# Autodesk Inventor assembly: SumpAssembly
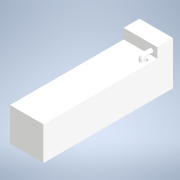
[picture p0: Inventor's stored thumbnail of the model, 180x180]
Saved by Autodesk Inventor 2022 (Build 260153000, 153)
## iProperties
Created: 2021-06-30
Part Number: SumpAssembly
Document SubType Name: Assembly
Designer: jamieson-bl
Author: jamieson-bl
## Documents named in this file (4)
- \\Mac\Home\Desktop\WinnipegPMTTestFacility\SumpAssembly.iam
- \\Mac\Home\Desktop\WinnipegPMTTestFacility\Sump_1SDB_Tub.ipt
- \\Mac\Home\Desktop\WinnipegPMTTestFacility\Sump Baffle Tub.ipt
- \\Mac\Home\Desktop\WinnipegPMTTestFacility\Sump Reservoir.ipt
## Components (4 placed, 3 different names)
1. Sump_1SDB_Tub:1 — Mate:1, Flush:1, Flush:2
2. Sump Baffle Tub:1 — Mate:1, Flush:1, Flush:2, Flush:3, Mate:2, Flush:5
3. Sump Reservoir:1 — Flush:3, Flush:4, Mate:2, Flush:5, Flush:6, Mate:3
4. Sump Reservoir:2 — Flush:4, Flush:6, Mate:3
## Relationships (9: Flush 6, Mate 3)
- Mate:1: Sump_1SDB_Tub:1 ↔ Sump Baffle Tub:1
- Flush:1: Sump_1SDB_Tub:1 ↔ Sump Baffle Tub:1
- Flush:2: Sump_1SDB_Tub:1 ↔ Sump Baffle Tub:1
- Flush:3: Sump Baffle Tub:1 ↔ Sump Reservoir:1
- Flush:4: Sump Reservoir:1 ↔ Sump Reservoir:2
- Mate:2: Sump Baffle Tub:1 ↔ Sump Reservoir:1
- Flush:5: Sump Baffle Tub:1 ↔ Sump Reservoir:1
- Flush:6: Sump Reservoir:1 ↔ Sump Reservoir:2
- Mate:3: Sump Reservoir:1 ↔ Sump Reservoir:2
